# Autodesk Inventor assembly: Pierna
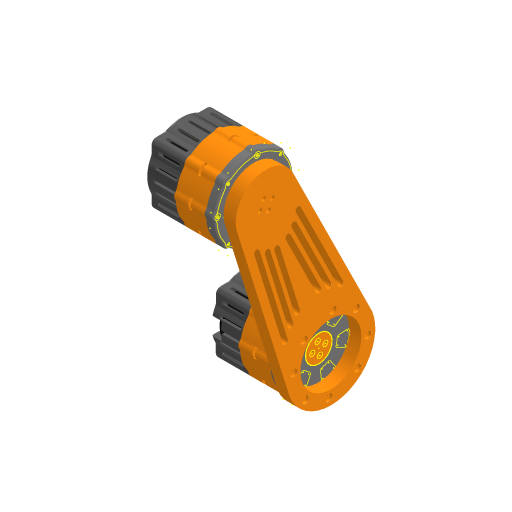
[picture p0: Inventor's stored thumbnail of the model, 512x512]
Saved by Autodesk Inventor 2024.3 (Build 283343000, 343)
## iProperties
Created: 2025-09-03
Part Number: Pierna
Document SubType Name: Assembly
Designer: danie
Author: danie
## Documents named in this file (3)
- C:\Users\danie\OneDrive\Documentos\Inventor\Motor_drive\Pierna.iam
- C:\Users\danie\OneDrive\Documentos\Inventor\Motor_drive\Ensamble.iam
- C:\Users\danie\OneDrive\Documentos\Inventor\Motor_drive\Link1.ipt
## Components (3 placed, 2 different names)
1. Ensamble:1 [sub-assembly] — Mate:2, Mate:3, Mate:4, Mate:6, Mate:10
2. Ensamble:2 [sub-assembly] — Mate:9, Mate:11
3. Link1:1 — Mate:6, Mate:9, Mate:10, Mate:11
## Relationships (7: Mate 7)
- Mate:2: Ensamble:1
- Mate:3: Ensamble:1
- Mate:4: Ensamble:1
- Mate:6: Ensamble:1 ↔ Link1:1
- Mate:9: Ensamble:2 ↔ Link1:1
- Mate:10: Ensamble:1 ↔ Link1:1
- Mate:11: Ensamble:2 ↔ Link1:1
